# Autodesk Inventor assembly: 4.1h_JulianR_Assembly
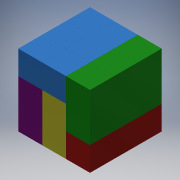
[picture p0: Inventor's stored thumbnail of the model, 180x180]
Saved by Autodesk Inventor 2016 (Build 200138000, 138)
## iProperties
Created: 2017-03-02
Part Number: 4.1h_JulianR_Assembly
Document SubType Name: Assembly
Designer: fhs-mgr
Author: fhs-mgr
## Documents named in this file (6)
- H:\IED 5th Inventor\4.1h_JulianR_Assembly.iam
- H:\IED 5th Inventor\4.1h_JulianR_Assemblypart1.iam
- H:\IED 5th Inventor\4.1h_JulianR_Assemblypart2.iam
- H:\IED 5th Inventor\4.1h_JulianR_Assemblypart3.iam
- H:\IED 5th Inventor\4.1h_JulianR_Assemblypart4.iam
- H:\IED 5th Inventor\4.1h_JulianR_Assemblypart5.iam
## Components (5 placed, 5 different names)
1. 4.1h_JulianR_Assemblypart1:1 [sub-assembly] — Mate:1, Mate:2, Mate:6
2. 4.1h_JulianR_Assemblypart2:1 [sub-assembly] — Mate:1, Mate:2, Mate:3, Mate:4, Mate:5
3. 4.1h_JulianR_Assemblypart3:1 [sub-assembly] — Mate:5, Mate:6, Mate:8
4. 4.1h_JulianR_Assemblypart4:1 [sub-assembly] — Mate:3, Mate:4, Mate:7
5. 4.1h_JulianR_Assemblypart5:1 [sub-assembly] — Mate:7, Mate:8
## Relationships (8: Mate 8)
- Mate:1: 4.1h_JulianR_Assemblypart1:1 ↔ 4.1h_JulianR_Assemblypart2:1
- Mate:2: 4.1h_JulianR_Assemblypart1:1 ↔ 4.1h_JulianR_Assemblypart2:1
- Mate:3: 4.1h_JulianR_Assemblypart2:1 ↔ 4.1h_JulianR_Assemblypart4:1
- Mate:4: 4.1h_JulianR_Assemblypart2:1 ↔ 4.1h_JulianR_Assemblypart4:1
- Mate:5: 4.1h_JulianR_Assemblypart2:1 ↔ 4.1h_JulianR_Assemblypart3:1
- Mate:6: 4.1h_JulianR_Assemblypart1:1 ↔ 4.1h_JulianR_Assemblypart3:1
- Mate:7: 4.1h_JulianR_Assemblypart4:1 ↔ 4.1h_JulianR_Assemblypart5:1
- Mate:8: 4.1h_JulianR_Assemblypart3:1 ↔ 4.1h_JulianR_Assemblypart5:1
